# Autodesk Inventor assembly: 42146-17
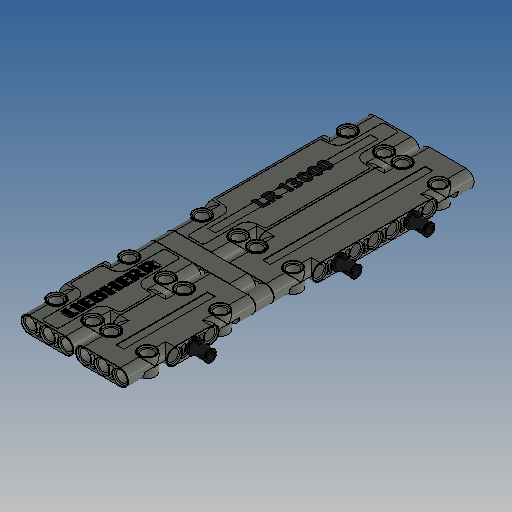
[picture p0: Inventor's stored thumbnail of the model, 512x512]
Saved by Autodesk Inventor 2025 (Build 290162010, 162A)
## iProperties
Created: 2024-11-18
Part Number: 42146-17
Material: Generisch
Document SubType Name: Assembly
Designer: hp.muther
Author: hp.muther
## Documents named in this file (9)
- D:\Inventor\Projekte\Muther\LEGO Technic\LEGO Technik - Raupenkran LR 13000 (42146)\42146-17.iam
- D:\Inventor\Projekte\Muther\LEGO Technic\LEGO Pieces\Paneelen\71709-DkBluishGray.ipt
- D:\Inventor\Projekte\Muther\LEGO Technic\LEGO Pieces\Pin's\2780-Black.ipt
- D:\Inventor\Projekte\Muther\LEGO Technic\LEGO Pieces\Pin's\6558-Blue.ipt
- D:\Inventor\Projekte\Muther\LEGO Technic\LEGO Pieces\Lochbalken\32316-DkBluishGray.ipt
- D:\Inventor\Projekte\Muther\LEGO Technic\LEGO Pieces\Rund\18654-DkBluishGray.ipt
- D:\Inventor\Projekte\Muther\LEGO Technic\LEGO Pieces\Paneelen\15458-DkBluishGray.ipt
- D:\Inventor\Projekte\Muther\LEGO Technic\LEGO Technik - Raupenkran LR 13000 (42146)\42146_15458_1.ipt
- D:\Inventor\Projekte\Muther\LEGO Technic\LEGO Technik - Raupenkran LR 13000 (42146)\42146_71709_1.ipt
## Components (17 placed, 8 different names)
1. 42146_71709_1:1 — Einfügen:1, Einfügen:2, Einfügen:6, Einfügen:7
2. 71709-DkBluishGray:2 — Einfügen:6, Passend:1, Passend:2, Einfügen:8, Einfügen:9, Einfügen:12
3. 2780-Black:1 — Einfügen:1, Passend:1
4. 2780-Black:2 — Einfügen:2
5. 6558-Blue:1 — Einfügen:4
6. 6558-Blue:2 — Einfügen:8, Passend:4
7. 6558-Blue:3 — Einfügen:3
8. 6558-Blue:4 — Einfügen:5, Passend:2
9. 2780-Black:3 — Einfügen:10
10. 2780-Black:4 — Einfügen:12
11. 2780-Black:5 — Einfügen:14
12. 2780-Black:6 — Einfügen:13
13. 2780-Black:7 — Einfügen:11, Passend:3
14. 32316-DkBluishGray:1 — Einfügen:3, Einfügen:4, Einfügen:5, Einfügen:7, Einfügen:16
15. 18654-DkBluishGray:1 — Einfügen:9
16. 15458-DkBluishGray:1 — Einfügen:13, Einfügen:14, Einfügen:15, Passend:3, Passend:4
17. 42146_15458_1:1 — Einfügen:10, Einfügen:11, Einfügen:15, Einfügen:16
## Relationships (20: Insert 16, Mate 4)
- Einfügen:1 [Insert]: 42146_71709_1:1 ↔ 2780-Black:1
- Einfügen:2 [Insert]: 42146_71709_1:1 ↔ 2780-Black:2
- Einfügen:3 [Insert]: 6558-Blue:3 ↔ 32316-DkBluishGray:1
- Einfügen:4 [Insert]: 6558-Blue:1 ↔ 32316-DkBluishGray:1
- Einfügen:5 [Insert]: 6558-Blue:4 ↔ 32316-DkBluishGray:1
- Einfügen:6 [Insert]: 42146_71709_1:1 ↔ 71709-DkBluishGray:2
- Passend:1 [Mate]: 71709-DkBluishGray:2 ↔ 2780-Black:1
- Einfügen:7 [Insert]: 42146_71709_1:1 ↔ 32316-DkBluishGray:1
- Passend:2 [Mate]: 71709-DkBluishGray:2 ↔ 6558-Blue:4
- Einfügen:8 [Insert]: 71709-DkBluishGray:2 ↔ 6558-Blue:2
- Einfügen:9 [Insert]: 71709-DkBluishGray:2 ↔ 18654-DkBluishGray:1
- Einfügen:10 [Insert]: 2780-Black:3 ↔ 42146_15458_1:1
- Einfügen:11 [Insert]: 2780-Black:7 ↔ 42146_15458_1:1
- Einfügen:12 [Insert]: 71709-DkBluishGray:2 ↔ 2780-Black:4
- Einfügen:13 [Insert]: 2780-Black:6 ↔ 15458-DkBluishGray:1
- Einfügen:14 [Insert]: 2780-Black:5 ↔ 15458-DkBluishGray:1
- Einfügen:15 [Insert]: 15458-DkBluishGray:1 ↔ 42146_15458_1:1
- Einfügen:16 [Insert]: 32316-DkBluishGray:1 ↔ 42146_15458_1:1
- Passend:3 [Mate]: 2780-Black:7 ↔ 15458-DkBluishGray:1
- Passend:4 [Mate]: 6558-Blue:2 ↔ 15458-DkBluishGray:1
